# Autodesk Inventor assembly: Assembly1
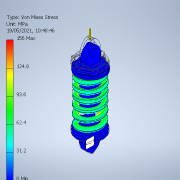
[picture p0: Inventor's stored thumbnail of the model, 180x180]
Saved by Autodesk Inventor 2020 (Build 240168000, 168)
## iProperties
Created: 2021-05-18
Part Number: Assembly1
Document SubType Name: Assembly
Designer: Andrew
Mass: 1975.57 g
Surface Area: 1069.87 cm^2
Volume: 442.668 cm^3
Density: 4.46287 g/cm^3
Author: Andrew
## Documents named in this file (11)
- C:\Users\Andrew\Documents\Works\Inventor\Shock2\Assembly1.iam
- C:\Users\Andrew\Documents\Works\Inventor\Shock2\Part1.ipt
- C:\Users\Andrew\Documents\Works\Inventor\Shock2\Part2.ipt
- C:\Users\Andrew\Documents\Works\Inventor\Shock2\Part3.ipt
- C:\Users\Andrew\Documents\Works\Inventor\Shock2\Part4.ipt
- C:\Users\Andrew\Documents\Works\Inventor\Shock2\Assembly1\AIP\FEA\dlz4j7jc0.fins
- C:\Users\Andrew\Documents\Works\Inventor\Shock2\Assembly1\AIP\FEA\dlz4j7jc0.fsat
- C:\Users\Andrew\Documents\Works\Inventor\Shock2\Assembly1\AIP\FEA\dlz4j7jc0.ftes
- C:\Users\Andrew\Documents\Works\Inventor\Shock2\Assembly1\AIP\FEA\dlz4j7jc0.fwiz
- C:\Users\Andrew\Documents\Works\Inventor\Shock2\Assembly1\AIP\FEA\dlz4j7jeo.fmsh
- C:\Users\Andrew\Documents\Works\Inventor\Shock2\Assembly1\AIP\FEA\dlz4j7jep.fres
## Components (4 placed, 4 different names)
1. Part1:1 — Mate:1, Mate:2, Mate:3, Mate:4, Mate:5
2. Part2:1 — Mate:3, Mate:4, Mate:6
3. Part3:1 — Mate:5, Mate:6, Mate:7
4. Part4:1 — Mate:1, Mate:2, Mate:7
## Relationships (7: Mate 7)
- Mate:1: Part1:1 ↔ Part4:1
- Mate:2: Part1:1 ↔ Part4:1
- Mate:3: Part1:1 ↔ Part2:1
- Mate:4: Part1:1 ↔ Part2:1
- Mate:5: Part1:1 ↔ Part3:1
- Mate:6: Part2:1 ↔ Part3:1
- Mate:7: Part3:1 ↔ Part4:1
## Named parameters: sa_0 = 0, sa_1 = -981, sa_2 = 0, sa_3 = 0, sa_4 = -65000, sa_5 = 0
note: some values were not read from the file. Shown as the stored number, unit unknown: "sa_0", "sa_1", "sa_2", "sa_3", "sa_4", "sa_5".
